# Autodesk Inventor assembly: gear_MIR
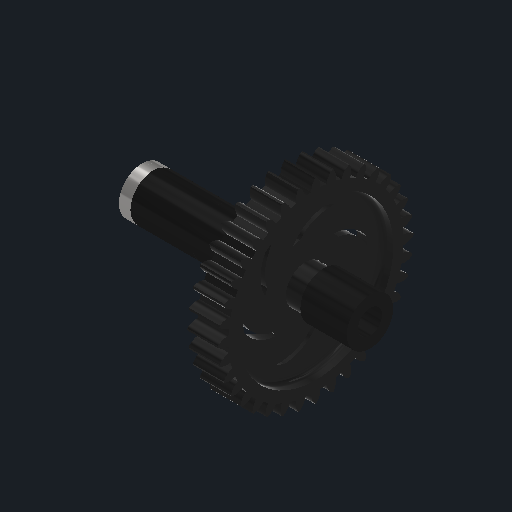
[picture p0: Inventor's stored thumbnail of the model, 512x512]
Saved by Autodesk Inventor 2024 (Build 280153000, 153)
## iProperties
Created: 2023-10-29
Part Number: gear_MIR
Document SubType Name: Assembly
Designer: avere
Author: Averey Ku
## Documents named in this file (8)
- C:\Users\avere\Documents\rbp_cad\zoomba_v0.1\chassis\mirrored_parts\gear_MIR.iam
- C:\Users\avere\Documents\rbp_cad\VEX-CAD-Inventor-1.41\Motion\Spacers\Spacer Nylon .375 OD\NSpacer .375 OD x .375.ipt
- C:\Users\avere\Documents\rbp_cad\VEX-CAD-Inventor-1.41\Motion\Spacers\Spacer Nylon .375 OD.ipt
- C:\Users\avere\Documents\rbp_cad\zoomba_v0.1\chassis\mirrored_parts\LS 36T Gear_MIR.ipt
- C:\Users\avere\Documents\rbp_cad\VEX-CAD-Inventor-1.41\Motion\Spacers\Spacer Nylon .375 OD\NSpacer .375 OD x .500.ipt
- C:\Users\avere\Documents\rbp_cad\VEX-CAD-Inventor-1.41\Motion\Spacers\Washer Steel\SWasher .375 OD x .062500.ipt
- C:\Users\avere\Documents\rbp_cad\VEX-CAD-Inventor-1.41\Motion\Spacers\Washer Steel.ipt
- C:\Users\avere\Documents\rbp_cad\VEX-CAD-Inventor-1.41\Motion\Spacers\Washer Steel\SWasher .375 OD x .031250.ipt
## Components (6 placed, 5 different names)
1. NSpacer .375 OD x .375:1 — Insert:1
2. LS 36T Gear_MIR:1 — Insert:1, Insert:5
3. NSpacer .375 OD x .500:2 — Insert:5, Insert:2
4. NSpacer .375 OD x .500:3 — Insert:2, Insert:4
5. SWasher .375 OD x .062500:1 — Insert:4, Insert:3
6. SWasher .375 OD x .031250:2 — Insert:3
## Relationships (5: Insert 5)
- Insert:1: NSpacer .375 OD x .375:1 ↔ LS 36T Gear_MIR:1
- Insert:5: LS 36T Gear_MIR:1 ↔ NSpacer .375 OD x .500:2
- Insert:2: NSpacer .375 OD x .500:2 ↔ NSpacer .375 OD x .500:3
- Insert:4: NSpacer .375 OD x .500:3 ↔ SWasher .375 OD x .062500:1
- Insert:3: SWasher .375 OD x .062500:1 ↔ SWasher .375 OD x .031250:2
